# Autodesk Inventor assembly: 10-06-05 Ansamblu nconector priza
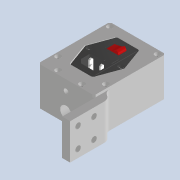
[picture p0: Inventor's stored thumbnail of the model, 180x180]
Saved by Autodesk Inventor 2020 (Build 240168000, 168)
## iProperties
Created: 2020-01-17
Part Number: 10-06-05 Ansamblu nconector priza
Document SubType Name: Assembly
Designer: iuliu
Author: iuliu
## Documents named in this file (4)
- Z:\I.A.B\Proiecte\0008 I.A.B 3D 2.1 Imprimanta aracet Metal\10 Mecanic\Ansamblu nconector priza.iam
- Z:\I.A.B\Proiecte\0008 I.A.B 3D 2.1 Imprimanta aracet Metal\10 Mecanic\0008-10-050 Suport conector cablu.ipt
- Z:\I.A.B\Proiecte\0008 I.A.B 3D 2.1 Imprimanta aracet Metal\20 Electric\0008-20-1006 Inlet Module Plug Fuse Switch Male Power Socket 10A 250V 3 Pin IEC320 C14.ipt
- Z:\I.A.B\Proiecte\0008 I.A.B 3D 2.1 Imprimanta aracet Metal\10 Mecanic\0008-10-051 Cutie Priza.ipt
## Components (3 placed, 3 different names)
1. 0008-10-050 Suport conector cablu:1 — Flush:1, Mate:1, Mate:2, Flush:4, Mate:3, Mate:4
2. 0008-20-1006 Inlet Module Plug Fuse Switch Male Power Socket 10A 250V 3 Pin IEC320 C14:1 — Flush:1, Mate:3, Mate:4
3. 0008-10-051 Cutie Priza:1 — Mate:1, Mate:2, Flush:4
## Relationships (6: Mate 4, Flush 2)
- Flush:1: 0008-10-050 Suport conector cablu:1 ↔ 0008-20-1006 Inlet Module Plug Fuse Switch Male Power Socket 10A 250V 3 Pin IEC320 C14:1
- Mate:1 (0.3 mm): 0008-10-050 Suport conector cablu:1 ↔ 0008-10-051 Cutie Priza:1
- Mate:2: 0008-10-050 Suport conector cablu:1 ↔ 0008-10-051 Cutie Priza:1
- Flush:4: 0008-10-050 Suport conector cablu:1 ↔ 0008-10-051 Cutie Priza:1
- Mate:3 (0.5 mm): 0008-10-050 Suport conector cablu:1 ↔ 0008-20-1006 Inlet Module Plug Fuse Switch Male Power Socket 10A 250V 3 Pin IEC320 C14:1
- Mate:4 (0.53 mm): 0008-10-050 Suport conector cablu:1 ↔ 0008-20-1006 Inlet Module Plug Fuse Switch Male Power Socket 10A 250V 3 Pin IEC320 C14:1
